# Autodesk Inventor assembly: station
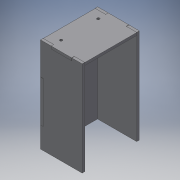
[picture p0: Inventor's stored thumbnail of the model, 180x180]
Saved by Autodesk Inventor 2017 (Build 210142000, 142)
## iProperties
Created: 2017-06-27
Part Number: station
Document SubType Name: Assembly
Designer: millerid
Author: millerid
## Documents named in this file (4)
- U:\Research\Swarms\RobotModel\StationModel\station.iam
- U:\Research\Swarms\RobotModel\StationModel\side.ipt
- U:\Research\Swarms\RobotModel\StationModel\back.ipt
- U:\Research\Swarms\RobotModel\StationModel\top.ipt
## Components (4 placed, 3 different names)
1. side:1 — Mate:2, Flush:2, Mate:3, Mate:4, Mate:5, Mate:8, Mate:9
2. side:2 — Mate:1, Flush:1, Mate:6, Mate:7
3. back:1 — Mate:4, Mate:5, Mate:6
4. top:1 — Mate:7, Mate:8, Mate:9
## Relationships (11: Mate 9, Flush 2)
- Mate:1: side:2
- Mate:2: side:1
- Flush:1: side:2
- Flush:2: side:1
- Mate:3: side:1
- Mate:4: side:1 ↔ back:1
- Mate:5: side:1 ↔ back:1
- Mate:6: side:2 ↔ back:1
- Mate:7: side:2 ↔ top:1
- Mate:8: side:1 ↔ top:1
- Mate:9: side:1 ↔ top:1
